# Autodesk Inventor assembly: GPSBackMountAssembly
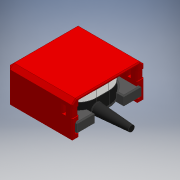
[picture p0: Inventor's stored thumbnail of the model, 180x180]
Saved by Autodesk Inventor 2019 (Build 230136000, 136)
## iProperties
Created: 2019-05-06
Part Number: GPSBackMountAssembly
Document SubType Name: Assembly
Designer: CASE-SMALL2
Author: CASE-SMALL2
## Documents named in this file (4)
- C:\Users\CASE-SMALL2\Google Drive\Kandidatarbete Rescuerunner\Drive-by-wire\Design docummentation\FRS (Front Rail System) _)\GPSBackMount\GPSBackMountAssembly.iam
- C:\Users\CASE-SMALL2\Google Drive\Kandidatarbete Rescuerunner\Drive-by-wire\Design docummentation\FRS (Front Rail System) _)\GPSBackMount\Platta.ipt
- C:\Users\CASE-SMALL2\Google Drive\Kandidatarbete Rescuerunner\Drive-by-wire\Design docummentation\FRS (Front Rail System) _)\FrontPanelMount\GPS_Antenna.ipt
- C:\Users\CASE-SMALL2\Google Drive\Kandidatarbete Rescuerunner\Drive-by-wire\Design docummentation\FRS (Front Rail System) _)\GPSBackMount\Top.ipt
## Components (3 placed, 3 different names)
1. Platta:1 — Flush:3
2. GPS_Antenna:1 — Flush:1, Flush:2, Flush:3
3. Top:1 — Flush:4, Mate:1, Flush:5
## Relationships (6: Flush 5, Mate 1)
- Flush:1: GPS_Antenna:1
- Flush:2: GPS_Antenna:1
- Flush:3 (3 mm): Platta:1 ↔ GPS_Antenna:1
- Flush:4: Top:1
- Mate:1: Top:1
- Flush:5 (5 mm): Top:1
